# Autodesk Inventor assembly: Bucket - 4 Rake
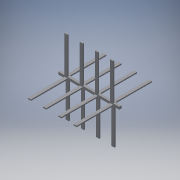
[picture p0: Inventor's stored thumbnail of the model, 180x180]
Saved by Autodesk Inventor 2016 (Build 200138000, 138)
## iProperties
Created: 2015-12-17
Part Number: Bucket - 4 Rake
Document SubType Name: Assembly
Designer: TimB
Author: TimB
## Documents named in this file (2)
- C:\Users\TimB\Documents\GitHub\phi_robotics\3d-models\FTC_Tetrix_KOP_Block_Party\Tim Bloot Designs\JAr JaR Bot\Bucket - 4 Rake.iam
- C:\Users\TimB\Documents\GitHub\phi_robotics\3d-models\FTC_Tetrix_KOP_Block_Party\Tim Bloot Designs\JAr JaR Bot\Bucket - Rake.ipt
## Components (4 placed, 1 different names)
1. Bucket - Rake:1 — Mate:1, Flush:1, Mate:2
2. Bucket - Rake:2 — Mate:1, Flush:1, Mate:2, Mate:3, Flush:2, Mate:4
3. Bucket - Rake:3 — Flush:3, Mate:5
4. Bucket - Rake:4 — Mate:3, Flush:2, Mate:4, Flush:3, Mate:5
## Relationships (8: Mate 5, Flush 3)
- Mate:1: Bucket - Rake:1 ↔ Bucket - Rake:2
- Flush:1: Bucket - Rake:1 ↔ Bucket - Rake:2
- Mate:2: Bucket - Rake:1 ↔ Bucket - Rake:2
- Mate:3: Bucket - Rake:2 ↔ Bucket - Rake:4
- Flush:2: Bucket - Rake:2 ↔ Bucket - Rake:4
- Mate:4: Bucket - Rake:2 ↔ Bucket - Rake:4
- Flush:3: Bucket - Rake:3 ↔ Bucket - Rake:4
- Mate:5: Bucket - Rake:3 ↔ Bucket - Rake:4
